# Autodesk Inventor assembly: LightPoint
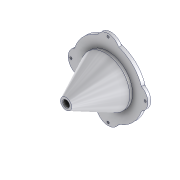
[picture p0: Inventor's stored thumbnail of the model, 180x180]
Saved by Autodesk Inventor 2020.3 (Build 243373010, 373A)
## iProperties
Created: 2020-12-04
Part Number: LightPoint
Document SubType Name: Assembly
Designer: Yusuf
Mass: 53.4206 g
Surface Area: 450.966 cm^2
Volume: 53.4206 cm^3
Density: 1 g/cm^3
Author: Yusuf
## Documents named in this file (5)
- C:\Users\Yusuf\Desktop\SunCollector\LightPoint.iam
- C:\Users\Yusuf\Desktop\SunCollector\LightPoint_LedStripMetal.ipt
- C:\Users\Yusuf\Desktop\SunCollector\LilghtPointLensHolder.ipt
- C:\Users\Yusuf\Desktop\SunCollector\LED3528SMD.ipt
- C:\Users\Yusuf\Desktop\SunCollector\Lens.ipt
## Components (23 placed, 4 different names)
1. LightPoint_LedStripMetal:1 — Mate:2, Mate:3, Mate:4, Mate:5
2. LilghtPointLensHolder:1 — Mate:2, Mate:3, Mate:6, Mate:7
3. Lens:1 — Mate:6, Mate:7
4. LED3528SMD:1 — Mate:4, Mate:5
5. LED3528SMD:2
6. LED3528SMD:3
7. LED3528SMD:4
8. LED3528SMD:5
9. LED3528SMD:6
10. LED3528SMD:7
11. LED3528SMD:8
12. LED3528SMD:9
13. LED3528SMD:10
14. LED3528SMD:11
15. LED3528SMD:12
16. LED3528SMD:13
17. LED3528SMD:14
18. LED3528SMD:15
19. LED3528SMD:16
20. LED3528SMD:17
21. LED3528SMD:18
22. LED3528SMD:19
23. LED3528SMD:20
## Component patterns: (20 elements, first: LED3528SMD:1)
## Relationships (6: Mate 6)
- Mate:2: LightPoint_LedStripMetal:1 ↔ LilghtPointLensHolder:1
- Mate:3: LightPoint_LedStripMetal:1 ↔ LilghtPointLensHolder:1
- Mate:4: LightPoint_LedStripMetal:1 ↔ LED3528SMD:1
- Mate:5: LightPoint_LedStripMetal:1 ↔ LED3528SMD:1
- Mate:6: LilghtPointLensHolder:1 ↔ Lens:1
- Mate:7: LilghtPointLensHolder:1 ↔ Lens:1
